# Autodesk Inventor assembly: ECU_SMD
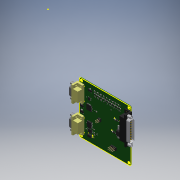
[picture p0: Inventor's stored thumbnail of the model, 180x180]
Saved by Autodesk Inventor 2019 (Build 230136000, 136)
## iProperties
Company: A Company
Created: 2019-03-11
Part Number: ECU_SMD
Description: KiCad electronic assembly
Document SubType Name: Assembly
Designer: A.SaleH
Authority: Unknown
Sending System: KiCad to STEP converter
Preprocessor: Open CASCADE STEP processor 6.9
Title: ECU_SMD.step
Author: An Author
## Documents named in this file (19)
- C:\Users\A.SaleH\Desktop\EV19\EV19\ECU_SMD\ECU_SMD.iam
- C:\Users\A.SaleH\Desktop\EV19\EV19\ECU_SMD\R_0805_2012Metric.iam
- C:\Users\A.SaleH\Desktop\EV19\EV19\ECU_SMD\DIP-4_W7.62mm.iam
- C:\Users\A.SaleH\Desktop\EV19\EV19\ECU_SMD\SOT-23-5.iam
- C:\Users\A.SaleH\Desktop\EV19\EV19\ECU_SMD\C_0805_2012Metric.iam
- C:\Users\A.SaleH\Desktop\EV19\EV19\ECU_SMD\C_1206_3216Metric.iam
- C:\Users\A.SaleH\Desktop\EV19\EV19\ECU_SMD\SOIC-16W_7.5x10.3mm_P1.27mm.iam
- C:\Users\A.SaleH\Desktop\EV19\EV19\ECU_SMD\SOIC-8_3.9x4.9mm_P1.27mm.iam
- C:\Users\A.SaleH\Desktop\EV19\EV19\ECU_SMD\SOT-223.iam
- C:\Users\A.SaleH\Desktop\EV19\EV19\ECU_SMD\LQFP-64_10x10mm_P0.5mm.iam
- C:\Users\A.SaleH\Desktop\EV19\EV19\ECU_SMD\SSO-8_6.8x5.9mm_P1.27mm_Clearance8mm.iam
- C:\Users\A.SaleH\Desktop\EV19\EV19\ECU_SMD\PinHeader_2x04_P2.54mm_Vertical.iam
- C:\Users\A.SaleH\Desktop\EV19\EV19\ECU_SMD\SOT-23.iam
- C:\Users\A.SaleH\Desktop\EV19\EV19\ECU_SMD\TO-220-3_Horizontal_TabDown.iam
- C:\Users\A.SaleH\Desktop\EV19\EV19\ECU_SMD\D_A-405_P10.16mm_Horizontal.iam
- C:\Users\A.SaleH\Desktop\EV19\EV19\ECU_SMD\PinHeader_2x02_P2.54mm_Vertical.iam
- C:\Users\A.SaleH\Desktop\EV19\EV19\ECU_SMD\COMPOUND.ipt
- C:\Users\A.SaleH\Documents\Inventor\Electric_EV\DB25RA_M.ipt
- C:\Users\A.SaleH\Documents\Inventor\Electric_EV\DB9RA_M.ipt
## Components (106 placed, 105 different names)
1. 2 [sub-assembly]
2. 4 [sub-assembly]
3. 6 [sub-assembly]
4. 8 [sub-assembly]
5. 9 [sub-assembly]
6. 10 [sub-assembly]
7. 11 [sub-assembly]
8. 12 [sub-assembly]
9. 13 [sub-assembly]
10. 14 [sub-assembly]
11. 15 [sub-assembly]
12. 16 [sub-assembly]
13. 17 [sub-assembly]
14. 18 [sub-assembly]
15. 20 [sub-assembly]
16. 21 [sub-assembly]
17. 22 [sub-assembly]
18. 23 [sub-assembly]
19. 24 [sub-assembly]
20. 25 [sub-assembly]
21. 26 [sub-assembly]
22. 27 [sub-assembly]
23. 28 [sub-assembly]
24. 29 [sub-assembly]
25. 30 [sub-assembly]
26. 31 [sub-assembly]
27. 32 [sub-assembly]
28. 33 [sub-assembly]
29. 34 [sub-assembly]
30. 35 [sub-assembly]
31. 36 [sub-assembly]
32. 37 [sub-assembly]
33. 38 [sub-assembly]
34. 39 [sub-assembly]
35. 40 [sub-assembly]
36. 41 [sub-assembly]
37. 42 [sub-assembly]
38. 43 [sub-assembly]
39. 44 [sub-assembly]
40. 45 [sub-assembly]
41. 46 [sub-assembly]
42. 47 [sub-assembly]
43. 48 [sub-assembly]
44. 49 [sub-assembly]
45. 50 [sub-assembly]
46. 51 [sub-assembly]
47. 52 [sub-assembly]
48. 53 [sub-assembly]
49. 54 [sub-assembly]
50. 55 [sub-assembly]
51. 56 [sub-assembly]
52. 57 [sub-assembly]
53. 58 [sub-assembly]
54. 59 [sub-assembly]
55. 60 [sub-assembly]
56. 61 [sub-assembly]
57. 62 [sub-assembly]
58. 63 [sub-assembly]
59. 64 [sub-assembly]
60. 65 [sub-assembly]
61. 66 [sub-assembly]
62. 67 [sub-assembly]
63. 68 [sub-assembly]
64. 70 [sub-assembly]
65. 72 [sub-assembly]
66. 74 [sub-assembly]
67. 75 [sub-assembly]
68. 77 [sub-assembly]
69. 78 [sub-assembly]
70. 79 [sub-assembly]
71. 80 [sub-assembly]
72. 81 [sub-assembly]
73. 82 [sub-assembly]
74. 83 [sub-assembly]
75. 84 [sub-assembly]
76. 85 [sub-assembly]
77. 86 [sub-assembly]
78. 87 [sub-assembly]
79. 88 [sub-assembly]
80. 89 [sub-assembly]
81. 90 [sub-assembly]
82. 91 [sub-assembly]
83. 92 [sub-assembly]
84. 93 [sub-assembly]
85. 94 [sub-assembly]
86. 95 [sub-assembly]
87. 96 [sub-assembly]
88. 97 [sub-assembly]
89. 98 [sub-assembly]
90. 99 [sub-assembly]
91. 100 [sub-assembly]
92. 102 [sub-assembly]
93. 103 [sub-assembly]
94. 105 [sub-assembly]
95. 107 [sub-assembly]
96. 109 [sub-assembly]
97. 110 [sub-assembly]
98. 111 [sub-assembly]
99. 113 [sub-assembly]
100. 114 [sub-assembly]
101. 115 [sub-assembly]
102. 117 [sub-assembly]
103. 118 — Mate:1, Mate:2, Mate:3, Mate:4, Mate:5, Mate:6
104. DB25RA_M:1 — Mate:1, Mate:2
105. DB9RA_M:1 — Mate:3, Mate:5
106. DB9RA_M:2 — Mate:4, Mate:6
## Relationships (6: Mate 6)
- Mate:1: 118 ↔ DB25RA_M:1
- Mate:2: 118 ↔ DB25RA_M:1
- Mate:3: 118 ↔ DB9RA_M:1
- Mate:4: 118 ↔ DB9RA_M:2
- Mate:5: 118 ↔ DB9RA_M:1
- Mate:6: 118 ↔ DB9RA_M:2
